# Autodesk Inventor assembly: Jig - Motor
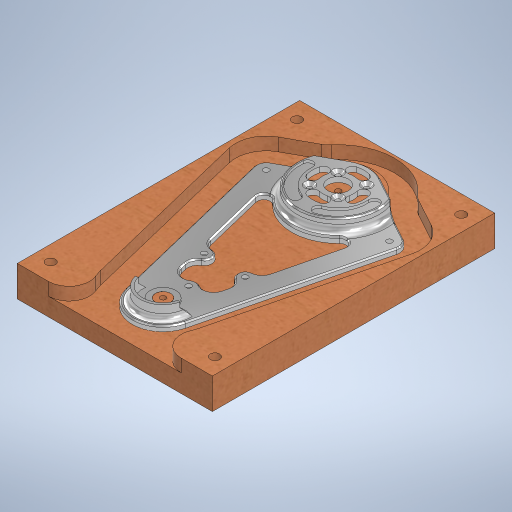
[picture p0: Inventor's stored thumbnail of the model, 512x512]
Saved by Autodesk Inventor 2023.2 (Build 272271000, 271)
## iProperties
Created: 2023-08-27
Part Number: Jig - Motor
Document SubType Name: Assembly
Designer: Nathan Cai
Author: Nathan Cai
## Documents named in this file (4)
- E:\Documents\Inventor\Law - V1.0\Vert - 1in\Jig - Motor.iam
- E:\Documents\Inventor\Law - V1.0\Vert - 1in\Upright - Motor.ipt
- E:\Documents\Inventor\Law - V1.0\Vert - 1in\Jig - Motor.ipt
- E:\Documents\Inventor\Law - V1.0\Vert - 1in\Upright - Blank.ipt
## Components (3 placed, 3 different names)
1. Upright - Motor:1 — Mate:1, Mate:2, Mate:3
2. Jig - Motor:1 — Mate:1, Mate:2, Mate:3, Mate:5, Mate:6, Mate:7
3. Upright - Blank:1 — Mate:5, Mate:6, Mate:7
## Relationships (6: Mate 6)
- Mate:1: Upright - Motor:1 ↔ Jig - Motor:1
- Mate:2: Upright - Motor:1 ↔ Jig - Motor:1
- Mate:3: Upright - Motor:1 ↔ Jig - Motor:1
- Mate:5: Jig - Motor:1 ↔ Upright - Blank:1
- Mate:6: Jig - Motor:1 ↔ Upright - Blank:1
- Mate:7: Jig - Motor:1 ↔ Upright - Blank:1
